# Autodesk Inventor assembly: bolt and nut assembly
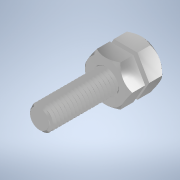
[picture p0: Inventor's stored thumbnail of the model, 180x180]
Saved by Autodesk Inventor 2022 (Build 260153000, 153)
## iProperties
Created: 2019-05-09
Part Number: bolt and nut assembly
Document SubType Name: Assembly
Designer: Administrator
Author: Administrator
## Documents named in this file (3)
- F:\Temp\Call of Duty - Black Ops\bolt-and-nut-39.snapshot.4\bolt and nut assembly.iam
- F:\Temp\Call of Duty - Black Ops\bolt-and-nut-39.snapshot.4\BOLT CREATION +  CREATED THREADS.ipt
- F:\Temp\Call of Duty - Black Ops\bolt-and-nut-39.snapshot.4\NUT CrEATION- NON STANDARD.ipt
## Components (2 placed, 2 different names)
1. BOLT CREATION +  CREATED THREADS:1 — Mate:1, Flush:1, Angle:1
2. NUT CrEATION- NON STANDARD:1 — Mate:1, Flush:1, Angle:1
## Relationships (3: Mate 1, Flush 1, Angle 1)
- Mate:1: BOLT CREATION +  CREATED THREADS:1 ↔ NUT CrEATION- NON STANDARD:1
- Flush:1: BOLT CREATION +  CREATED THREADS:1 ↔ NUT CrEATION- NON STANDARD:1
- Angle:1 (0 deg): BOLT CREATION +  CREATED THREADS:1 ↔ NUT CrEATION- NON STANDARD:1
